# Autodesk Inventor assembly: Сборка1
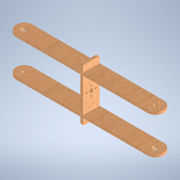
[picture p0: Inventor's stored thumbnail of the model, 180x180]
Saved by Autodesk Inventor 2020.1 (Build 241239000, 239)
## iProperties
Created: 2021-08-12
Part Number: Сборка1
Document SubType Name: Assembly
Designer: Ni3na
Mass: 25.1888 g
Surface Area: 253.767 cm^2
Volume: 39.9823 cm^3
Density: 0.63 g/cm^3
Author: Ni3na
## Documents named in this file (3)
- D:\GitHub\avatar-kvantoriada\3D\Сборка1.iam
- D:\GitHub\avatar-kvantoriada\3D\Деталь1.ipt
- D:\GitHub\avatar-kvantoriada\3D\Деталь2.ipt
## Components (3 placed, 2 different names)
1. Деталь2:1 — Жесткий:1, Жесткий:2
2. Деталь1:3 — Жесткий:1
3. Деталь1:4 — Жесткий:2
## Relationships (2: WeldJoint 2)
- Жесткий:1 [WeldJoint]: Деталь2:1 ↔ Деталь1:3
- Жесткий:2 [WeldJoint]: Деталь2:1 ↔ Деталь1:4
